# Autodesk Inventor assembly: Assembly1
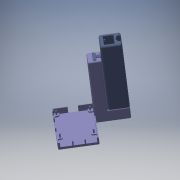
[picture p0: Inventor's stored thumbnail of the model, 180x180]
Saved by Autodesk Inventor 2018 (Build 220112000, 112)
## iProperties
Created: 2017-11-10
Part Number: Assembly1
Document SubType Name: Assembly
Designer: kameo
Author: kameo
## Documents named in this file (7)
- C:\Users\kameo\Documents\IoTToothbrush\CAD\Assembly1.iam
- C:\Users\kameo\Documents\IoTToothbrush\CAD\Toothbrush.ipt
- C:\Users\kameo\Documents\IoTToothbrush\CAD\Female Header -X- TH 2.54mm Pitch\Female Header 2.54mm Pitch 1x8.ipt
- C:\Users\kameo\Documents\IoTToothbrush\CAD\Female Header -X- TH 2.54mm Pitch.ipt
- C:\Users\kameo\Documents\IoTToothbrush\CAD\BaseStation.ipt
- C:\Users\kameo\Documents\IoTToothbrush\CAD\Male Header -X- TH 2.54mm Pitch\Male Header 2.54mm Pitch 1x8.ipt
- C:\Users\kameo\Documents\IoTToothbrush\CAD\Male Header -X- TH 2.54mm Pitch.ipt
## Components (4 placed, 4 different names)
1. Toothbrush:1 — Mate:1, Flush:1, Mate:2, Mate:3, Mate:4
2. Female Header 2.54mm Pitch 1x8:1 — Mate:1, Flush:1, Mate:2
3. BaseStation:1 — Mate:3, Mate:4, Flush:2, Mate:5, Mate:6
4. Male Header 2.54mm Pitch 1x8:1 — Flush:2, Mate:5, Mate:6
## Relationships (8: Mate 6, Flush 2)
- Mate:1: Toothbrush:1 ↔ Female Header 2.54mm Pitch 1x8:1
- Flush:1: Toothbrush:1 ↔ Female Header 2.54mm Pitch 1x8:1
- Mate:2: Toothbrush:1 ↔ Female Header 2.54mm Pitch 1x8:1
- Mate:3: Toothbrush:1 ↔ BaseStation:1
- Mate:4: Toothbrush:1 ↔ BaseStation:1
- Flush:2: BaseStation:1 ↔ Male Header 2.54mm Pitch 1x8:1
- Mate:5: BaseStation:1 ↔ Male Header 2.54mm Pitch 1x8:1
- Mate:6: BaseStation:1 ↔ Male Header 2.54mm Pitch 1x8:1
